# Autodesk Inventor assembly: clamp_mechanism
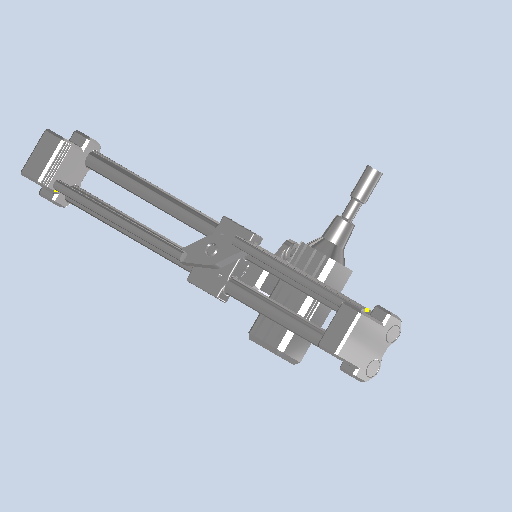
[picture p0: Inventor's stored thumbnail of the model, 512x512]
Saved by Autodesk Inventor 2023 (Build 270158000, 158)
## iProperties
Created: 2023-11-21
Part Number: clamp_mechanism
Document SubType Name: Assembly
Designer: Beatrice
Author: Beatrice
## Documents named in this file (9)
- E:\WORKSPACE_2\wheel_changing_assignment\clamp_mechanism.iam
- E:\WORKSPACE_2\wheel_changing_assignment\robot_tool_arm.ipt
- E:\WORKSPACE_2\wheel_changing_assignment\robotic_arrm tool slider.ipt
- E:\WORKSPACE_2\wheel_changing_assignment\robotic_wheel_clamp.ipt
- E:\WORKSPACE_2\wheel_changing_assignment\robotic_wheel_clamp_MIR.ipt
- E:\WORKSPACE_2\wheel_changing_assignment\clamp_mechanism.ipt
- E:\WORKSPACE_2\wheel_changing_assignment\clamp_rod.ipt
- E:\WORKSPACE_2\wheel_changing_assignment\screwdriver.ipt
- E:\WORKSPACE_2\wheel_changing_assignment\lagnut_screw.ipt
## Components (9 placed, 8 different names)
1. robot_tool_arm:1 — Mate:1, Mate:2, Flush:5, Mate:5, Mate:13, Mate:15
2. robotic_arrm tool slider:1 — Mate:1, Mate:2, Mate:3, Mate:4, Flush:3, Flush:4
3. robotic_wheel_clamp:1 — Flush:1, Flush:2, Flush:4
4. robotic_wheel_clamp_MIR:1 — Flush:1, Flush:2, Mate:3, Mate:4, Flush:3, Mate:11
5. clamp_mechanism:1 — Flush:5, Mate:5, Mate:6, Mate:7, Mate:8, Mate:9
6. clamp_rod:1 — Mate:6, Mate:7, Mate:11
7. clamp_rod:3 — Mate:8, Mate:9
8. screwdriver:1 — Mate:12, Mate:13, Mate:14, Mate:15
9. lagnut_screw:1 — Mate:12, Mate:14
## Relationships (19: Mate 14, Flush 5)
- Mate:1: robot_tool_arm:1 ↔ robotic_arrm tool slider:1
- Mate:2 (0.8 mm): robot_tool_arm:1 ↔ robotic_arrm tool slider:1
- Flush:1: robotic_wheel_clamp:1 ↔ robotic_wheel_clamp_MIR:1
- Flush:2: robotic_wheel_clamp:1 ↔ robotic_wheel_clamp_MIR:1
- Mate:3: robotic_arrm tool slider:1 ↔ robotic_wheel_clamp_MIR:1
- Mate:4: robotic_arrm tool slider:1 ↔ robotic_wheel_clamp_MIR:1
- Flush:3: robotic_arrm tool slider:1 ↔ robotic_wheel_clamp_MIR:1
- Flush:4: robotic_arrm tool slider:1 ↔ robotic_wheel_clamp:1
- Flush:5: robot_tool_arm:1 ↔ clamp_mechanism:1
- Mate:5: robot_tool_arm:1 ↔ clamp_mechanism:1
- Mate:6: clamp_mechanism:1 ↔ clamp_rod:1
- Mate:7: clamp_mechanism:1 ↔ clamp_rod:1
- Mate:8: clamp_mechanism:1 ↔ clamp_rod:3
- Mate:9: clamp_mechanism:1 ↔ clamp_rod:3
- Mate:11: robotic_wheel_clamp_MIR:1 ↔ clamp_rod:1
- Mate:12: screwdriver:1 ↔ lagnut_screw:1
- Mate:13: robot_tool_arm:1 ↔ screwdriver:1
- Mate:14: screwdriver:1 ↔ lagnut_screw:1
- Mate:15 (0.5 mm): robot_tool_arm:1 ↔ screwdriver:1
